# Autodesk Inventor assembly: Box Arm
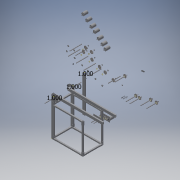
[picture p0: Inventor's stored thumbnail of the model, 180x180]
Saved by Autodesk Inventor 2018 (Build 220112000, 112)
## iProperties
Created: 2019-01-16
Part Number: Box Arm
Document SubType Name: Assembly
Designer: Gabriel
Author: Gabriel
## Documents named in this file (20)
- C:\Users\Gabriel\Documents\GitHub\2019CAD\Drivebase Box Arm\Box Arm.iam
- C:\Users\Gabriel\Documents\GitHub\2019CAD\Drivebase Box Arm\30in 1x1 Beam.ipt
- C:\Users\Gabriel\Documents\GitHub\2019CAD\Drivebase Box Arm\25in 1x1 Beam.ipt
- C:\Users\Gabriel\Documents\GitHub\2019CAD\Drivebase Box Arm\17in 1x1 Beam.ipt
- C:\Users\Gabriel\Documents\GitHub\2019CAD\Drivebase Box Arm\23in 1x1 Beam.ipt
- C:\Users\Gabriel\Documents\GitHub\2019CAD\Drivebase Box Arm\L gusset.ipt
- C:\Users\Gabriel\Documents\GitHub\2019CAD\Drivebase Box Arm\34.48in Arm Bea.ipt
- C:\Users\Gabriel\Documents\GitHub\2019CAD\Drivebase Box Arm\0_500_ID_x_1_125_OD_x_0_313_WD_Flanged_Bearing_217-2731.ipt
- C:\Users\Gabriel\Documents\GitHub\2019CAD\Drivebase Box Arm\_72t_Aluminum_Plate_Sprocket_25_Chain_1-1_8_Bearing_Bore_217-2627.ipt
- C:\Users\Gabriel\Documents\GitHub\2019CAD\Drivebase Box Arm\Hex Hub.ipt
- C:\Users\Gabriel\Documents\GitHub\2019CAD\Drivebase Box Arm\0.5in Hex Shaft.ipt
- C:\Users\Gabriel\Documents\GitHub\2019CAD\Drivebase Box Arm\half_inch_collar.ipt
- C:\Users\Gabriel\Documents\GitHub\2019CAD\Drivebase Box Arm\1_2_Acetal_Spacer_-_1_2_Hex_217-3261.ipt
- C:\Users\Gabriel\Documents\GitHub\2019CAD\Drivebase Box Arm\_16t_Aluminum_Hub_Sprocket_25_Chain_1_2_Hex_Bore_217-2642.ipt
- C:\Users\Gabriel\Documents\GitHub\2019CAD\Drivebase Box Arm\18t_Aluminum_Spur_Gear_20_DP_1_2_Hex_Bore_217-3209.ipt
- C:\Users\Gabriel\Documents\GitHub\2019CAD\Drivebase Box Arm\am-0150 Toughbox Large Output Gear.ipt
- C:\Users\Gabriel\Documents\GitHub\2019CAD\Drivebase Box Arm\Mini_CIM_Motor_217-3371.ipt
- C:\Users\Gabriel\Documents\GitHub\2019CAD\Drivebase Box Arm\9T_Steel_Spur_Gear_20_DP_10T_Center_Distance_CIM_Motor_217-6335.ipt
- C:\Users\Gabriel\Documents\GitHub\2019CAD\Drivebase Box Arm\ARm Gearbox Plate.ipt
- C:\Users\Gabriel\Documents\GitHub\2019CAD\Drivebase Box Arm\1_16_Acetal_Spacer_-_1_2_Hex_217-3257.ipt
## Components (159 placed, 19 different names)
1. 30in 1x1 Beam:1 — Mate:13, Mate:14, Mate:37, Mate:38, Mate:74, Mate:75, Mate:83, Mate:84, Mate:98, Mate:99, Mate:101, Mate:102, Mate:103, Mate:104
2. 30in 1x1 Beam:2 — Mate:11, Mate:12, Mate:39, Mate:40, Mate:73, Mate:76, Mate:86, Mate:87, Mate:95, Mate:96, Mate:105, Mate:106, Mate:107, Mate:108
3. 25in 1x1 Beam:1 — Mate:57, Mate:58, Mate:59, Mate:60, Mate:65, Mate:66, Mate:90, Mate:91
4. 25in 1x1 Beam:2 — Mate:61, Mate:62, Mate:63, Mate:64, Mate:67, Mate:68, Mate:93, Mate:94
5. 25in 1x1 Beam:3 — Mate:29, Mate:30, Mate:53, Mate:54, Mate:97
6. 25in 1x1 Beam:4 — Mate:31, Mate:32, Mate:55, Mate:56, Mate:100
7. 17in 1x1 Beam:1 — Mate:69, Mate:70, Mate:71, Mate:72
8. 17in 1x1 Beam:2 — Mate:21, Mate:22, Mate:23, Mate:24
9. 23in 1x1 Beam:1 — Mate:43, Mate:44, Mate:49, Mate:50, Mate:88, Mate:92
10. 23in 1x1 Beam:2 — Mate:47, Mate:48, Mate:51, Mate:52, Mate:85, Mate:89
11. L gusset:1 — Mate:53, Mate:54, Mate:63, Mate:64
12. L gusset:4 — Mate:49, Mate:50, Mate:61, Mate:62
13. L gusset:5 — Mate:51, Mate:52, Mate:57, Mate:58
14. L gusset:7 — Mate:11, Mate:12, Mate:23, Mate:24
15. L gusset:9 — Mate:13, Mate:14, Mate:21, Mate:22
16. L gusset:11 — Mate:31, Mate:32, Mate:74, Mate:75
17. L gusset:12 — Mate:29, Mate:30, Mate:73, Mate:76
18. L gusset:13 — Mate:43, Mate:44
19. L gusset:14 — Mate:47, Mate:48
20. L gusset:15 — Mate:39, Mate:40, Mate:77, Mate:80
21. L gusset:16 — Mate:37, Mate:38, Mate:78, Mate:79
22. L gusset:17 — Mate:55, Mate:56, Mate:59, Mate:60
23. L gusset:18 — Mate:67, Mate:68, Mate:69, Mate:70
24. L gusset:19 — Mate:65, Mate:66, Mate:71, Mate:72
25. 17in 1x1 Beam:3 — Mate:77, Mate:78, Mate:79, Mate:80
26. 34.48in Arm Bea:2 — Mate:109, Mate:110, Mate:145
27. 0_500_ID_x_1_125_OD_x_0_313_WD_Flanged_Bearing_217-2731:1 — Mate:103, Mate:104, Mate:139, Mate:140, Mate:149
28. 0_500_ID_x_1_125_OD_x_0_313_WD_Flanged_Bearing_217-2731:2 — Mate:107, Mate:108, Mate:126, Mate:152
29. 0_500_ID_x_1_125_OD_x_0_313_WD_Flanged_Bearing_217-2731:3
30. 0_500_ID_x_1_125_OD_x_0_313_WD_Flanged_Bearing_217-2731:5 — Mate:101, Mate:102, Mate:143
31. 0_500_ID_x_1_125_OD_x_0_313_WD_Flanged_Bearing_217-2731:8 — Mate:105, Mate:106, Mate:122
32. L gusset:20 — Mate:92, Mate:93, Mate:94
33. L gusset:21 — Mate:89, Mate:90, Mate:91
34. L gusset:22 — Mate:98, Mate:99, Mate:100
35. L gusset:23 — Mate:95, Mate:96, Mate:97
36. L gusset:24 — Mate:83, Mate:84, Mate:85
37. L gusset:25 — Mate:86, Mate:87, Mate:88
38. _72t_Aluminum_Plate_Sprocket_25_Chain_1-1_8_Bearing_Bore_217-2627:2 — Mate:120, Mate:121, Mate:138
39. Hex Hub:2 — Mate:109, Mate:110, Mate:111, Mate:112, Mate:113, Mate:114, Mate:115
40. Hex Hub:3 — Mate:116, Mate:117, Mate:118, Mate:120, Mate:121, Mate:122, Mate:138
41. 0.5in Hex Shaft:2 — Mate:114, Mate:115, Mate:116, Mate:117, Mate:123, Mate:124, Mate:125, Mate:150, Mate:151
42. half_inch_collar:1 — Mate:145
43. half_inch_collar:2 — Mate:146
44. half_inch_collar:4 — Mate:127
45. 1_2_Acetal_Spacer_-_1_2_Hex_217-3261:1 — Mate:123, Mate:124, Mate:125, Mate:126, Mate:127
46. 1_2_Acetal_Spacer_-_1_2_Hex_217-3261:3 — Mate:111, Mate:112, Mate:113, Mate:118
47. 34.48in Arm Bea:3 — Mate:128, Mate:146
48. _72t_Aluminum_Plate_Sprocket_25_Chain_1-1_8_Bearing_Bore_217-2627:3 — Mate:137
49. Hex Hub:4 — Mate:134, Mate:135, Mate:136, Mate:137, Mate:139, Mate:140
50. Hex Hub:5 — Mate:128, Mate:129, Mate:130, Mate:133
51. 0.5in Hex Shaft:3 — Mate:129, Mate:130, Mate:131, Mate:132, Mate:134, Mate:135, Mate:141, Mate:142, Mate:147, Mate:148
52. half_inch_collar:5 — Mate:144
53. 1_2_Acetal_Spacer_-_1_2_Hex_217-3261:7 — Mate:141, Mate:142, Mate:143, Mate:144
54. 1_2_Acetal_Spacer_-_1_2_Hex_217-3261:8 — Mate:131, Mate:132, Mate:133, Mate:136
55. 1_2_Acetal_Spacer_-_1_2_Hex_217-3261:9 — Mate:147, Mate:148, Mate:149
56. 1_2_Acetal_Spacer_-_1_2_Hex_217-3261:10 — Mate:150, Mate:151, Mate:152
57. 30in 1x1 Beam:3
58. _16t_Aluminum_Hub_Sprocket_25_Chain_1_2_Hex_Bore_217-2642:1
59. 0.5in Hex Shaft:4
60. 18t_Aluminum_Spur_Gear_20_DP_1_2_Hex_Bore_217-3209:1
61. am-0150 Toughbox Large Output Gear:1
62. half_inch_collar:6
63. Mini_CIM_Motor_217-3371:1
64. _16t_Aluminum_Hub_Sprocket_25_Chain_1_2_Hex_Bore_217-2642:2
65. 0.5in Hex Shaft:5
66. 18t_Aluminum_Spur_Gear_20_DP_1_2_Hex_Bore_217-3209:2
67. am-0150 Toughbox Large Output Gear:2
68. half_inch_collar:7
69. Mini_CIM_Motor_217-3371:2 — Mate:165, Mate:166, Mate:167, Mate:168
70. _16t_Aluminum_Hub_Sprocket_25_Chain_1_2_Hex_Bore_217-2642:3
71. 0.5in Hex Shaft:6 — Mate:169, Mate:170, Mate:171, Mate:172, Mate:173
72. 18t_Aluminum_Spur_Gear_20_DP_1_2_Hex_Bore_217-3209:3 — Mate:172, Mate:173, Mate:174
73. am-0150 Toughbox Large Output Gear:3 — Mate:169, Mate:170, Mate:171, Mate:174
74. half_inch_collar:8
75. Mini_CIM_Motor_217-3371:3
76. _16t_Aluminum_Hub_Sprocket_25_Chain_1_2_Hex_Bore_217-2642:4
77. half_inch_collar:9
78. Mini_CIM_Motor_217-3371:4
79. _16t_Aluminum_Hub_Sprocket_25_Chain_1_2_Hex_Bore_217-2642:5
80. 0.5in Hex Shaft:8
81. 18t_Aluminum_Spur_Gear_20_DP_1_2_Hex_Bore_217-3209:5
82. am-0150 Toughbox Large Output Gear:5
83. half_inch_collar:10
84. Mini_CIM_Motor_217-3371:5
85. _16t_Aluminum_Hub_Sprocket_25_Chain_1_2_Hex_Bore_217-2642:6
86. 0.5in Hex Shaft:9
87. 18t_Aluminum_Spur_Gear_20_DP_1_2_Hex_Bore_217-3209:6
88. am-0150 Toughbox Large Output Gear:6
89. half_inch_collar:11
90. Mini_CIM_Motor_217-3371:6
91. _16t_Aluminum_Hub_Sprocket_25_Chain_1_2_Hex_Bore_217-2642:7
92. 0.5in Hex Shaft:10
93. 18t_Aluminum_Spur_Gear_20_DP_1_2_Hex_Bore_217-3209:7
94. am-0150 Toughbox Large Output Gear:7
95. half_inch_collar:12
96. Mini_CIM_Motor_217-3371:7
97. _16t_Aluminum_Hub_Sprocket_25_Chain_1_2_Hex_Bore_217-2642:8
98. 0.5in Hex Shaft:11
99. 18t_Aluminum_Spur_Gear_20_DP_1_2_Hex_Bore_217-3209:8
100. am-0150 Toughbox Large Output Gear:8
101. half_inch_collar:13
102. Mini_CIM_Motor_217-3371:8
103. 9T_Steel_Spur_Gear_20_DP_10T_Center_Distance_CIM_Motor_217-6335:1
104. 9T_Steel_Spur_Gear_20_DP_10T_Center_Distance_CIM_Motor_217-6335:2 — Mate:167, Mate:168
105. ARm Gearbox Plate:1 — Mate:159, Mate:160, Mate:161, Mate:162, Mate:163, Mate:164
106. ARm Gearbox Plate:2 — Mate:153, Mate:154, Mate:155, Mate:156, Mate:157, Mate:158, Mate:165, Mate:166
107. 0_500_ID_x_1_125_OD_x_0_313_WD_Flanged_Bearing_217-2731:9 — Mate:153, Mate:156, Mate:200, Mate:201
108. 0_500_ID_x_1_125_OD_x_0_313_WD_Flanged_Bearing_217-2731:10 — Mate:155, Mate:158, Mate:272
109. 0_500_ID_x_1_125_OD_x_0_313_WD_Flanged_Bearing_217-2731:11 — Mate:154, Mate:157, Mate:241
110. 0_500_ID_x_1_125_OD_x_0_313_WD_Flanged_Bearing_217-2731:12 — Mate:160, Mate:163
111. 0_500_ID_x_1_125_OD_x_0_313_WD_Flanged_Bearing_217-2731:13 — Mate:159, Mate:164
112. 0_500_ID_x_1_125_OD_x_0_313_WD_Flanged_Bearing_217-2731:14 — Mate:161, Mate:162
113. 0.5in Hex Shaft:12 — Mate:188, Mate:189
114. 18t_Aluminum_Spur_Gear_20_DP_1_2_Hex_Bore_217-3209:9
115. am-0150 Toughbox Large Output Gear:9 — Mate:190
116. 1_16_Acetal_Spacer_-_1_2_Hex_217-3257:1
117. 1_16_Acetal_Spacer_-_1_2_Hex_217-3257:2 — Mate:188, Mate:189, Mate:190
118. 1_16_Acetal_Spacer_-_1_2_Hex_217-3257:3
119. 1_16_Acetal_Spacer_-_1_2_Hex_217-3257:4
120. 1_16_Acetal_Spacer_-_1_2_Hex_217-3257:5
121. 1_16_Acetal_Spacer_-_1_2_Hex_217-3257:6
122. 1_16_Acetal_Spacer_-_1_2_Hex_217-3257:7
123. 1_16_Acetal_Spacer_-_1_2_Hex_217-3257:8
124. 1_16_Acetal_Spacer_-_1_2_Hex_217-3257:9
125. 1_16_Acetal_Spacer_-_1_2_Hex_217-3257:10
126. 0.5in Hex Shaft:13 — Mate:199
127. 18t_Aluminum_Spur_Gear_20_DP_1_2_Hex_Bore_217-3209:10 — Mate:199
128. am-0150 Toughbox Large Output Gear:10
129. 1_16_Acetal_Spacer_-_1_2_Hex_217-3257:11 — Mate:200, Mate:201
130. 0.5in Hex Shaft:14 — Mate:210, Mate:211, Mate:212
131. 18t_Aluminum_Spur_Gear_20_DP_1_2_Hex_Bore_217-3209:11 — Mate:210
132. am-0150 Toughbox Large Output Gear:11 — Mate:240
133. 1_2_Acetal_Spacer_-_1_2_Hex_217-3261:11
134. 1_2_Acetal_Spacer_-_1_2_Hex_217-3261:12 — Mate:242, Mate:243, Mate:244, Mate:247
135. 1_2_Acetal_Spacer_-_1_2_Hex_217-3261:13
136. 1_2_Acetal_Spacer_-_1_2_Hex_217-3261:14 — Mate:245, Mate:246, Mate:247, Mate:272
137. 1_2_Acetal_Spacer_-_1_2_Hex_217-3261:15
138. 1_2_Acetal_Spacer_-_1_2_Hex_217-3261:16 — Mate:211, Mate:212, Mate:240, Mate:241
139. 0.5in Hex Shaft:15 — Mate:242, Mate:243, Mate:245, Mate:246
140. 18t_Aluminum_Spur_Gear_20_DP_1_2_Hex_Bore_217-3209:12
141. am-0150 Toughbox Large Output Gear:12 — Mate:244
142. 0.5in Hex Shaft:16
143. 18t_Aluminum_Spur_Gear_20_DP_1_2_Hex_Bore_217-3209:13
144. am-0150 Toughbox Large Output Gear:13
145. 1_16_Acetal_Spacer_-_1_2_Hex_217-3257:14
146. 0.5in Hex Shaft:17
147. 18t_Aluminum_Spur_Gear_20_DP_1_2_Hex_Bore_217-3209:14
148. am-0150 Toughbox Large Output Gear:14
149. 1_16_Acetal_Spacer_-_1_2_Hex_217-3257:15
150. 1_2_Acetal_Spacer_-_1_2_Hex_217-3261:17
151. 1_2_Acetal_Spacer_-_1_2_Hex_217-3261:18
152. 0.5in Hex Shaft:18
153. 18t_Aluminum_Spur_Gear_20_DP_1_2_Hex_Bore_217-3209:15
154. am-0150 Toughbox Large Output Gear:15
155. 1_2_Acetal_Spacer_-_1_2_Hex_217-3261:19
156. 1_2_Acetal_Spacer_-_1_2_Hex_217-3261:20
157. 0.5in Hex Shaft:19
158. 18t_Aluminum_Spur_Gear_20_DP_1_2_Hex_Bore_217-3209:16
159. am-0150 Toughbox Large Output Gear:16
## Relationships (227: Mate 227)
- Mate:11: 30in 1x1 Beam:2 ↔ L gusset:7
- Mate:12: 30in 1x1 Beam:2 ↔ L gusset:7
- Mate:13: 30in 1x1 Beam:1 ↔ L gusset:9
- Mate:14: 30in 1x1 Beam:1 ↔ L gusset:9
- Mate:21: 17in 1x1 Beam:2 ↔ L gusset:9
- Mate:22: 17in 1x1 Beam:2 ↔ L gusset:9
- Mate:23: 17in 1x1 Beam:2 ↔ L gusset:7
- Mate:24: 17in 1x1 Beam:2 ↔ L gusset:7
- Mate:29: 25in 1x1 Beam:3 ↔ L gusset:12
- Mate:30: 25in 1x1 Beam:3 ↔ L gusset:12
- Mate:31: 25in 1x1 Beam:4 ↔ L gusset:11
- Mate:32: 25in 1x1 Beam:4 ↔ L gusset:11
- Mate:37: 30in 1x1 Beam:1 ↔ L gusset:16
- Mate:38: 30in 1x1 Beam:1 ↔ L gusset:16
- Mate:39: 30in 1x1 Beam:2 ↔ L gusset:15
- Mate:40: 30in 1x1 Beam:2 ↔ L gusset:15
- Mate:43: 23in 1x1 Beam:1 ↔ L gusset:13
- Mate:44: 23in 1x1 Beam:1 ↔ L gusset:13
- Mate:47: 23in 1x1 Beam:2 ↔ L gusset:14
- Mate:48: 23in 1x1 Beam:2 ↔ L gusset:14
- Mate:49: 23in 1x1 Beam:1 ↔ L gusset:4
- Mate:50: 23in 1x1 Beam:1 ↔ L gusset:4
- Mate:51: 23in 1x1 Beam:2 ↔ L gusset:5
- Mate:52: 23in 1x1 Beam:2 ↔ L gusset:5
- Mate:53: 25in 1x1 Beam:3 ↔ L gusset:1
- Mate:54: 25in 1x1 Beam:3 ↔ L gusset:1
- Mate:55: 25in 1x1 Beam:4 ↔ L gusset:17
- Mate:56: 25in 1x1 Beam:4 ↔ L gusset:17
- Mate:57: 25in 1x1 Beam:1 ↔ L gusset:5
- Mate:58: 25in 1x1 Beam:1 ↔ L gusset:5
- Mate:59: 25in 1x1 Beam:1 ↔ L gusset:17
- Mate:60: 25in 1x1 Beam:1 ↔ L gusset:17
- Mate:61: 25in 1x1 Beam:2 ↔ L gusset:4
- Mate:62: 25in 1x1 Beam:2 ↔ L gusset:4
- Mate:63: 25in 1x1 Beam:2 ↔ L gusset:1
- Mate:64: 25in 1x1 Beam:2 ↔ L gusset:1
- Mate:65: 25in 1x1 Beam:1 ↔ L gusset:19
- Mate:66: 25in 1x1 Beam:1 ↔ L gusset:19
- Mate:67: 25in 1x1 Beam:2 ↔ L gusset:18
- Mate:68: 25in 1x1 Beam:2 ↔ L gusset:18
- Mate:69: 17in 1x1 Beam:1 ↔ L gusset:18
- Mate:70: 17in 1x1 Beam:1 ↔ L gusset:18
- Mate:71: 17in 1x1 Beam:1 ↔ L gusset:19
- Mate:72: 17in 1x1 Beam:1 ↔ L gusset:19
- Mate:73: 30in 1x1 Beam:2 ↔ L gusset:12
- Mate:74: 30in 1x1 Beam:1 ↔ L gusset:11
- Mate:75: 30in 1x1 Beam:1 ↔ L gusset:11
- Mate:76: 30in 1x1 Beam:2 ↔ L gusset:12
- Mate:77: L gusset:15 ↔ 17in 1x1 Beam:3
- Mate:78: L gusset:16 ↔ 17in 1x1 Beam:3
- Mate:79: L gusset:16 ↔ 17in 1x1 Beam:3
- Mate:80: L gusset:15 ↔ 17in 1x1 Beam:3
- Mate:83: 30in 1x1 Beam:1 ↔ L gusset:24
- Mate:84: 30in 1x1 Beam:1 ↔ L gusset:24
- Mate:85: 23in 1x1 Beam:2 ↔ L gusset:24
- Mate:86: 30in 1x1 Beam:2 ↔ L gusset:25
- Mate:87: 30in 1x1 Beam:2 ↔ L gusset:25
- Mate:88: 23in 1x1 Beam:1 ↔ L gusset:25
- Mate:89: 23in 1x1 Beam:2 ↔ L gusset:21
- Mate:90: 25in 1x1 Beam:1 ↔ L gusset:21
- Mate:91: 25in 1x1 Beam:1 ↔ L gusset:21
- Mate:92: 23in 1x1 Beam:1 ↔ L gusset:20
- Mate:93: 25in 1x1 Beam:2 ↔ L gusset:20
- Mate:94: 25in 1x1 Beam:2 ↔ L gusset:20
- Mate:95: 30in 1x1 Beam:2 ↔ L gusset:23
- Mate:96: 30in 1x1 Beam:2 ↔ L gusset:23
- Mate:97: 25in 1x1 Beam:3 ↔ L gusset:23
- Mate:98: 30in 1x1 Beam:1 ↔ L gusset:22
- Mate:99: 30in 1x1 Beam:1 ↔ L gusset:22
- Mate:100: 25in 1x1 Beam:4 ↔ L gusset:22
- Mate:101: 30in 1x1 Beam:1 ↔ 0_500_ID_x_1_125_OD_x_0_313_WD_Flanged_Bearing_217-2731:5
- Mate:102: 30in 1x1 Beam:1 ↔ 0_500_ID_x_1_125_OD_x_0_313_WD_Flanged_Bearing_217-2731:5
- Mate:103: 30in 1x1 Beam:1 ↔ 0_500_ID_x_1_125_OD_x_0_313_WD_Flanged_Bearing_217-2731:1
- Mate:104: 30in 1x1 Beam:1 ↔ 0_500_ID_x_1_125_OD_x_0_313_WD_Flanged_Bearing_217-2731:1
- Mate:105: 30in 1x1 Beam:2 ↔ 0_500_ID_x_1_125_OD_x_0_313_WD_Flanged_Bearing_217-2731:8
- Mate:106: 30in 1x1 Beam:2 ↔ 0_500_ID_x_1_125_OD_x_0_313_WD_Flanged_Bearing_217-2731:8
- Mate:107: 30in 1x1 Beam:2 ↔ 0_500_ID_x_1_125_OD_x_0_313_WD_Flanged_Bearing_217-2731:2
- Mate:108: 30in 1x1 Beam:2 ↔ 0_500_ID_x_1_125_OD_x_0_313_WD_Flanged_Bearing_217-2731:2
- Mate:109: 34.48in Arm Bea:2 ↔ Hex Hub:2
- Mate:110: 34.48in Arm Bea:2 ↔ Hex Hub:2
- Mate:111: Hex Hub:2 ↔ 1_2_Acetal_Spacer_-_1_2_Hex_217-3261:3
- Mate:112: Hex Hub:2 ↔ 1_2_Acetal_Spacer_-_1_2_Hex_217-3261:3
- Mate:113: Hex Hub:2 ↔ 1_2_Acetal_Spacer_-_1_2_Hex_217-3261:3
- Mate:114: Hex Hub:2 ↔ 0.5in Hex Shaft:2
- Mate:115: Hex Hub:2 ↔ 0.5in Hex Shaft:2
- Mate:116: Hex Hub:3 ↔ 0.5in Hex Shaft:2
- Mate:117: Hex Hub:3 ↔ 0.5in Hex Shaft:2
- Mate:118: Hex Hub:3 ↔ 1_2_Acetal_Spacer_-_1_2_Hex_217-3261:3
- Mate:120: _72t_Aluminum_Plate_Sprocket_25_Chain_1-1_8_Bearing_Bore_217-2627:2 ↔ Hex Hub:3
- Mate:121: _72t_Aluminum_Plate_Sprocket_25_Chain_1-1_8_Bearing_Bore_217-2627:2 ↔ Hex Hub:3
- Mate:122: 0_500_ID_x_1_125_OD_x_0_313_WD_Flanged_Bearing_217-2731:8 ↔ Hex Hub:3
- Mate:123: 0.5in Hex Shaft:2 ↔ 1_2_Acetal_Spacer_-_1_2_Hex_217-3261:1
- Mate:124: 0.5in Hex Shaft:2 ↔ 1_2_Acetal_Spacer_-_1_2_Hex_217-3261:1
- Mate:125: 0.5in Hex Shaft:2 ↔ 1_2_Acetal_Spacer_-_1_2_Hex_217-3261:1
- Mate:126: 0_500_ID_x_1_125_OD_x_0_313_WD_Flanged_Bearing_217-2731:2 ↔ 1_2_Acetal_Spacer_-_1_2_Hex_217-3261:1
- Mate:127: half_inch_collar:4 ↔ 1_2_Acetal_Spacer_-_1_2_Hex_217-3261:1
- Mate:128: 34.48in Arm Bea:3 ↔ Hex Hub:5
- Mate:129: Hex Hub:5 ↔ 0.5in Hex Shaft:3
- Mate:130: Hex Hub:5 ↔ 0.5in Hex Shaft:3
- Mate:131: 0.5in Hex Shaft:3 ↔ 1_2_Acetal_Spacer_-_1_2_Hex_217-3261:8
- Mate:132: 0.5in Hex Shaft:3 ↔ 1_2_Acetal_Spacer_-_1_2_Hex_217-3261:8
- Mate:133: Hex Hub:5 ↔ 1_2_Acetal_Spacer_-_1_2_Hex_217-3261:8
- Mate:134: Hex Hub:4 ↔ 0.5in Hex Shaft:3
- Mate:135: Hex Hub:4 ↔ 0.5in Hex Shaft:3
- Mate:136: Hex Hub:4 ↔ 1_2_Acetal_Spacer_-_1_2_Hex_217-3261:8
- Mate:137: _72t_Aluminum_Plate_Sprocket_25_Chain_1-1_8_Bearing_Bore_217-2627:3 ↔ Hex Hub:4
- Mate:138: _72t_Aluminum_Plate_Sprocket_25_Chain_1-1_8_Bearing_Bore_217-2627:2 ↔ Hex Hub:3
- Mate:139: 0_500_ID_x_1_125_OD_x_0_313_WD_Flanged_Bearing_217-2731:1 ↔ Hex Hub:4
- Mate:140: 0_500_ID_x_1_125_OD_x_0_313_WD_Flanged_Bearing_217-2731:1 ↔ Hex Hub:4
- Mate:141: 0.5in Hex Shaft:3 ↔ 1_2_Acetal_Spacer_-_1_2_Hex_217-3261:7
- Mate:142: 0.5in Hex Shaft:3 ↔ 1_2_Acetal_Spacer_-_1_2_Hex_217-3261:7
- Mate:143: 0_500_ID_x_1_125_OD_x_0_313_WD_Flanged_Bearing_217-2731:5 ↔ 1_2_Acetal_Spacer_-_1_2_Hex_217-3261:7
- Mate:144: half_inch_collar:5 ↔ 1_2_Acetal_Spacer_-_1_2_Hex_217-3261:7
- Mate:145: 34.48in Arm Bea:2 ↔ half_inch_collar:1
- Mate:146: half_inch_collar:2 ↔ 34.48in Arm Bea:3
- Mate:147: 0.5in Hex Shaft:3 ↔ 1_2_Acetal_Spacer_-_1_2_Hex_217-3261:9
- Mate:148: 0.5in Hex Shaft:3 ↔ 1_2_Acetal_Spacer_-_1_2_Hex_217-3261:9
- Mate:149: 0_500_ID_x_1_125_OD_x_0_313_WD_Flanged_Bearing_217-2731:1 ↔ 1_2_Acetal_Spacer_-_1_2_Hex_217-3261:9
- Mate:150: 0.5in Hex Shaft:2 ↔ 1_2_Acetal_Spacer_-_1_2_Hex_217-3261:10
- Mate:151: 0.5in Hex Shaft:2 ↔ 1_2_Acetal_Spacer_-_1_2_Hex_217-3261:10
- Mate:152: 0_500_ID_x_1_125_OD_x_0_313_WD_Flanged_Bearing_217-2731:2 ↔ 1_2_Acetal_Spacer_-_1_2_Hex_217-3261:10
- Mate:153: ARm Gearbox Plate:2 ↔ 0_500_ID_x_1_125_OD_x_0_313_WD_Flanged_Bearing_217-2731:9
- Mate:154: ARm Gearbox Plate:2 ↔ 0_500_ID_x_1_125_OD_x_0_313_WD_Flanged_Bearing_217-2731:11
- Mate:155: ARm Gearbox Plate:2 ↔ 0_500_ID_x_1_125_OD_x_0_313_WD_Flanged_Bearing_217-2731:10
- Mate:156: ARm Gearbox Plate:2 ↔ 0_500_ID_x_1_125_OD_x_0_313_WD_Flanged_Bearing_217-2731:9
- Mate:157: ARm Gearbox Plate:2 ↔ 0_500_ID_x_1_125_OD_x_0_313_WD_Flanged_Bearing_217-2731:11
- Mate:158: ARm Gearbox Plate:2 ↔ 0_500_ID_x_1_125_OD_x_0_313_WD_Flanged_Bearing_217-2731:10
- Mate:159: ARm Gearbox Plate:1 ↔ 0_500_ID_x_1_125_OD_x_0_313_WD_Flanged_Bearing_217-2731:13
- Mate:160: ARm Gearbox Plate:1 ↔ 0_500_ID_x_1_125_OD_x_0_313_WD_Flanged_Bearing_217-2731:12
- Mate:161: ARm Gearbox Plate:1 ↔ 0_500_ID_x_1_125_OD_x_0_313_WD_Flanged_Bearing_217-2731:14
- Mate:162: ARm Gearbox Plate:1 ↔ 0_500_ID_x_1_125_OD_x_0_313_WD_Flanged_Bearing_217-2731:14
- Mate:163: ARm Gearbox Plate:1 ↔ 0_500_ID_x_1_125_OD_x_0_313_WD_Flanged_Bearing_217-2731:12
- Mate:164: ARm Gearbox Plate:1 ↔ 0_500_ID_x_1_125_OD_x_0_313_WD_Flanged_Bearing_217-2731:13
- Mate:165: Mini_CIM_Motor_217-3371:2 ↔ ARm Gearbox Plate:2
- Mate:166: Mini_CIM_Motor_217-3371:2 ↔ ARm Gearbox Plate:2
- Mate:167: Mini_CIM_Motor_217-3371:2 ↔ 9T_Steel_Spur_Gear_20_DP_10T_Center_Distance_CIM_Motor_217-6335:2
- Mate:168: Mini_CIM_Motor_217-3371:2 ↔ 9T_Steel_Spur_Gear_20_DP_10T_Center_Distance_CIM_Motor_217-6335:2
- Mate:169: 0.5in Hex Shaft:6 ↔ am-0150 Toughbox Large Output Gear:3
- Mate:170: 0.5in Hex Shaft:6 ↔ am-0150 Toughbox Large Output Gear:3
- Mate:171: 0.5in Hex Shaft:6 ↔ am-0150 Toughbox Large Output Gear:3
- Mate:172: 0.5in Hex Shaft:6 ↔ 18t_Aluminum_Spur_Gear_20_DP_1_2_Hex_Bore_217-3209:3
- Mate:173: 0.5in Hex Shaft:6 ↔ 18t_Aluminum_Spur_Gear_20_DP_1_2_Hex_Bore_217-3209:3
- Mate:174: 18t_Aluminum_Spur_Gear_20_DP_1_2_Hex_Bore_217-3209:3 ↔ am-0150 Toughbox Large Output Gear:3
- [Mate]: 0.5in Hex Shaft:12 ↔ am-0150 Toughbox Large Output Gear:9
- [Mate]: 0.5in Hex Shaft:12 ↔ am-0150 Toughbox Large Output Gear:9
- [Mate]: 0.5in Hex Shaft:12 ↔ am-0150 Toughbox Large Output Gear:9
- [Mate]: 0.5in Hex Shaft:12 ↔ 18t_Aluminum_Spur_Gear_20_DP_1_2_Hex_Bore_217-3209:9
- [Mate]: 18t_Aluminum_Spur_Gear_20_DP_1_2_Hex_Bore_217-3209:9 ↔ am-0150 Toughbox Large Output Gear:9
- Mate:188: 0.5in Hex Shaft:12 ↔ 1_16_Acetal_Spacer_-_1_2_Hex_217-3257:2
- Mate:189: 0.5in Hex Shaft:12 ↔ 1_16_Acetal_Spacer_-_1_2_Hex_217-3257:2
- Mate:190: am-0150 Toughbox Large Output Gear:9 ↔ 1_16_Acetal_Spacer_-_1_2_Hex_217-3257:2
- [Mate]: 0.5in Hex Shaft:13 ↔ am-0150 Toughbox Large Output Gear:10
- [Mate]: 0.5in Hex Shaft:13 ↔ am-0150 Toughbox Large Output Gear:10
- [Mate]: 0.5in Hex Shaft:13 ↔ am-0150 Toughbox Large Output Gear:10
- [Mate]: 0.5in Hex Shaft:13 ↔ 18t_Aluminum_Spur_Gear_20_DP_1_2_Hex_Bore_217-3209:10
- [Mate]: 18t_Aluminum_Spur_Gear_20_DP_1_2_Hex_Bore_217-3209:10 ↔ am-0150 Toughbox Large Output Gear:10
- [Mate]: 0.5in Hex Shaft:13 ↔ 1_16_Acetal_Spacer_-_1_2_Hex_217-3257:11
- [Mate]: 0.5in Hex Shaft:13 ↔ 1_16_Acetal_Spacer_-_1_2_Hex_217-3257:11
- [Mate]: am-0150 Toughbox Large Output Gear:10 ↔ 1_16_Acetal_Spacer_-_1_2_Hex_217-3257:11
- Mate:199: 0.5in Hex Shaft:13 ↔ 18t_Aluminum_Spur_Gear_20_DP_1_2_Hex_Bore_217-3209:10
- Mate:200: 0_500_ID_x_1_125_OD_x_0_313_WD_Flanged_Bearing_217-2731:9 ↔ 1_16_Acetal_Spacer_-_1_2_Hex_217-3257:11
- Mate:201: 0_500_ID_x_1_125_OD_x_0_313_WD_Flanged_Bearing_217-2731:9 ↔ 1_16_Acetal_Spacer_-_1_2_Hex_217-3257:11
- [Mate]: 0.5in Hex Shaft:14 ↔ am-0150 Toughbox Large Output Gear:11
- [Mate]: 0.5in Hex Shaft:14 ↔ am-0150 Toughbox Large Output Gear:11
- [Mate]: 0.5in Hex Shaft:14 ↔ am-0150 Toughbox Large Output Gear:11
- [Mate]: 0.5in Hex Shaft:14 ↔ 18t_Aluminum_Spur_Gear_20_DP_1_2_Hex_Bore_217-3209:11
- [Mate]: 18t_Aluminum_Spur_Gear_20_DP_1_2_Hex_Bore_217-3209:11 ↔ am-0150 Toughbox Large Output Gear:11
- Mate:210: 0.5in Hex Shaft:14 ↔ 18t_Aluminum_Spur_Gear_20_DP_1_2_Hex_Bore_217-3209:11
- Mate:211: 0.5in Hex Shaft:14 ↔ 1_2_Acetal_Spacer_-_1_2_Hex_217-3261:16
- Mate:212: 0.5in Hex Shaft:14 ↔ 1_2_Acetal_Spacer_-_1_2_Hex_217-3261:16
- [Mate]: 0.5in Hex Shaft:15 ↔ am-0150 Toughbox Large Output Gear:12
- [Mate]: 0.5in Hex Shaft:15 ↔ am-0150 Toughbox Large Output Gear:12
- [Mate]: 0.5in Hex Shaft:15 ↔ am-0150 Toughbox Large Output Gear:12
- [Mate]: 0.5in Hex Shaft:15 ↔ 18t_Aluminum_Spur_Gear_20_DP_1_2_Hex_Bore_217-3209:12
- [Mate]: 18t_Aluminum_Spur_Gear_20_DP_1_2_Hex_Bore_217-3209:12 ↔ am-0150 Toughbox Large Output Gear:12
- [Mate]: 0.5in Hex Shaft:15 ↔ 18t_Aluminum_Spur_Gear_20_DP_1_2_Hex_Bore_217-3209:12
- [Mate]: 0.5in Hex Shaft:16 ↔ am-0150 Toughbox Large Output Gear:13
- [Mate]: 0.5in Hex Shaft:16 ↔ am-0150 Toughbox Large Output Gear:13
- [Mate]: 0.5in Hex Shaft:16 ↔ am-0150 Toughbox Large Output Gear:13
- [Mate]: 0.5in Hex Shaft:16 ↔ 18t_Aluminum_Spur_Gear_20_DP_1_2_Hex_Bore_217-3209:13
- [Mate]: 18t_Aluminum_Spur_Gear_20_DP_1_2_Hex_Bore_217-3209:13 ↔ am-0150 Toughbox Large Output Gear:13
- [Mate]: 0.5in Hex Shaft:16 ↔ 1_16_Acetal_Spacer_-_1_2_Hex_217-3257:14
- [Mate]: 0.5in Hex Shaft:16 ↔ 1_16_Acetal_Spacer_-_1_2_Hex_217-3257:14
- [Mate]: am-0150 Toughbox Large Output Gear:13 ↔ 1_16_Acetal_Spacer_-_1_2_Hex_217-3257:14
- [Mate]: 0.5in Hex Shaft:16 ↔ 18t_Aluminum_Spur_Gear_20_DP_1_2_Hex_Bore_217-3209:13
- [Mate]: 0.5in Hex Shaft:17 ↔ am-0150 Toughbox Large Output Gear:14
- [Mate]: 0.5in Hex Shaft:17 ↔ am-0150 Toughbox Large Output Gear:14
- [Mate]: 0.5in Hex Shaft:17 ↔ am-0150 Toughbox Large Output Gear:14
- [Mate]: 0.5in Hex Shaft:17 ↔ 18t_Aluminum_Spur_Gear_20_DP_1_2_Hex_Bore_217-3209:14
- [Mate]: 18t_Aluminum_Spur_Gear_20_DP_1_2_Hex_Bore_217-3209:14 ↔ am-0150 Toughbox Large Output Gear:14
- [Mate]: 0.5in Hex Shaft:17 ↔ 1_16_Acetal_Spacer_-_1_2_Hex_217-3257:15
- [Mate]: 0.5in Hex Shaft:17 ↔ 1_16_Acetal_Spacer_-_1_2_Hex_217-3257:15
- [Mate]: am-0150 Toughbox Large Output Gear:14 ↔ 1_16_Acetal_Spacer_-_1_2_Hex_217-3257:15
- [Mate]: 0.5in Hex Shaft:17 ↔ 18t_Aluminum_Spur_Gear_20_DP_1_2_Hex_Bore_217-3209:14
- Mate:240: am-0150 Toughbox Large Output Gear:11 ↔ 1_2_Acetal_Spacer_-_1_2_Hex_217-3261:16
- Mate:241: 0_500_ID_x_1_125_OD_x_0_313_WD_Flanged_Bearing_217-2731:11 ↔ 1_2_Acetal_Spacer_-_1_2_Hex_217-3261:16
- Mate:242: 1_2_Acetal_Spacer_-_1_2_Hex_217-3261:12 ↔ 0.5in Hex Shaft:15
- Mate:243: 1_2_Acetal_Spacer_-_1_2_Hex_217-3261:12 ↔ 0.5in Hex Shaft:15
- Mate:244: 1_2_Acetal_Spacer_-_1_2_Hex_217-3261:12 ↔ am-0150 Toughbox Large Output Gear:12
- Mate:245: 1_2_Acetal_Spacer_-_1_2_Hex_217-3261:14 ↔ 0.5in Hex Shaft:15
- Mate:246: 1_2_Acetal_Spacer_-_1_2_Hex_217-3261:14 ↔ 0.5in Hex Shaft:15
- Mate:247: 1_2_Acetal_Spacer_-_1_2_Hex_217-3261:12 ↔ 1_2_Acetal_Spacer_-_1_2_Hex_217-3261:14
- [Mate]: 0.5in Hex Shaft:18 ↔ am-0150 Toughbox Large Output Gear:15
- [Mate]: 0.5in Hex Shaft:18 ↔ am-0150 Toughbox Large Output Gear:15
- [Mate]: 0.5in Hex Shaft:18 ↔ am-0150 Toughbox Large Output Gear:15
- [Mate]: 0.5in Hex Shaft:18 ↔ 18t_Aluminum_Spur_Gear_20_DP_1_2_Hex_Bore_217-3209:15
- [Mate]: 18t_Aluminum_Spur_Gear_20_DP_1_2_Hex_Bore_217-3209:15 ↔ am-0150 Toughbox Large Output Gear:15
- [Mate]: 0.5in Hex Shaft:18 ↔ 18t_Aluminum_Spur_Gear_20_DP_1_2_Hex_Bore_217-3209:15
- [Mate]: 1_2_Acetal_Spacer_-_1_2_Hex_217-3261:17 ↔ 0.5in Hex Shaft:18
- [Mate]: 1_2_Acetal_Spacer_-_1_2_Hex_217-3261:17 ↔ 0.5in Hex Shaft:18
- [Mate]: 1_2_Acetal_Spacer_-_1_2_Hex_217-3261:17 ↔ am-0150 Toughbox Large Output Gear:15
- [Mate]: 1_2_Acetal_Spacer_-_1_2_Hex_217-3261:18 ↔ 0.5in Hex Shaft:18
- [Mate]: 1_2_Acetal_Spacer_-_1_2_Hex_217-3261:18 ↔ 0.5in Hex Shaft:18
- [Mate]: 1_2_Acetal_Spacer_-_1_2_Hex_217-3261:17 ↔ 1_2_Acetal_Spacer_-_1_2_Hex_217-3261:18
- [Mate]: 0.5in Hex Shaft:19 ↔ am-0150 Toughbox Large Output Gear:16
- [Mate]: 0.5in Hex Shaft:19 ↔ am-0150 Toughbox Large Output Gear:16
- [Mate]: 0.5in Hex Shaft:19 ↔ am-0150 Toughbox Large Output Gear:16
- [Mate]: 0.5in Hex Shaft:19 ↔ 18t_Aluminum_Spur_Gear_20_DP_1_2_Hex_Bore_217-3209:16
- [Mate]: 18t_Aluminum_Spur_Gear_20_DP_1_2_Hex_Bore_217-3209:16 ↔ am-0150 Toughbox Large Output Gear:16
- [Mate]: 0.5in Hex Shaft:19 ↔ 18t_Aluminum_Spur_Gear_20_DP_1_2_Hex_Bore_217-3209:16
- [Mate]: 1_2_Acetal_Spacer_-_1_2_Hex_217-3261:19 ↔ 0.5in Hex Shaft:19
- [Mate]: 1_2_Acetal_Spacer_-_1_2_Hex_217-3261:19 ↔ 0.5in Hex Shaft:19
- [Mate]: 1_2_Acetal_Spacer_-_1_2_Hex_217-3261:19 ↔ am-0150 Toughbox Large Output Gear:16
- [Mate]: 1_2_Acetal_Spacer_-_1_2_Hex_217-3261:20 ↔ 0.5in Hex Shaft:19
- [Mate]: 1_2_Acetal_Spacer_-_1_2_Hex_217-3261:20 ↔ 0.5in Hex Shaft:19
- [Mate]: 1_2_Acetal_Spacer_-_1_2_Hex_217-3261:19 ↔ 1_2_Acetal_Spacer_-_1_2_Hex_217-3261:20
- Mate:272: 0_500_ID_x_1_125_OD_x_0_313_WD_Flanged_Bearing_217-2731:10 ↔ 1_2_Acetal_Spacer_-_1_2_Hex_217-3261:14
## Named parameters: d203_d194 = 0 mm, d204_d195 = 0 mm, d205_d196 = 0 mm, d206_d198 = 0 mm, d207_d199 = 0 mm, d212_d203_d194 = 0 mm, d213_d204_d195 = 0 mm, d214_d205_d196 = 0 mm, d215_d206_d198 = 0 mm, d216_d207_d199 = 0 mm, d217_d209 = 0 mm, d218_d210 = 0 mm, d219_d211 = 0 mm, d223_d203_d194 = 0 mm, d224_d204_d195 = 0 mm, d225_d205_d196 = 0 mm, d226_d206_d198 = 0 mm, d227_d207_d199 = 0 mm, d235_d223_d203_d194 = 0 mm, d236_d224_d204_d195 = 0 mm, d237_d225_d205_d196 = 0 mm, d238_d226_d206_d198 = 0 mm, d239_d227_d207_d199 = 0 mm, d243_d232 = 0 mm, d244_d223_d203_d194 = 0 mm, d245_d224_d204_d195 = 0 mm, d246_d225_d205_d196 = 0 mm, d247_d226_d206_d198 = 0 mm, d248_d227_d207_d199 = 0 mm, d249_d228_d209 = 0 mm, d250_d229_d210 = 0 mm, d251_d230_d211 = 0 mm, d252_d232 = 0 mm, d253_d223_d203_d194 = 0 mm, d254_d224_d204_d195 = 0 mm, d255_d225_d205_d196 = 0 mm, d256_d226_d206_d198 = 0 mm, d257_d227_d207_d199 = 0 mm, d258_d228_d209 = 0 mm, d259_d229_d210 = 0 mm, d260_d230_d211 = 0 mm, d261_d232 = 0 mm, d270_d235_d223_d203_d194 = 0 mm, d271_d236_d224_d204_d195 = 0 mm, d272_d237_d225_d205_d196 = 0 mm, d273_d238_d226_d206_d198 = 0 mm, d274_d239_d227_d207_d199 = 0 mm, d275_d243_d232 = 0 mm, d276_d264 = 0 mm, d277_d265 = 0 mm, d278_d266 = 0 mm, d279_d267 = 0 mm, d280_d268 = 0 mm, d281_d269 = 0 mm, d282_d235_d223_d203_d194 = 0 mm, d283_d236_d224_d204_d195 = 0 mm, d284_d237_d225_d205_d196 = 0 mm, d285_d238_d226_d206_d198 = 0 mm, d286_d239_d227_d207_d199 = 0 mm, d287_d243_d232 = 0 mm, d288_d264 = 0 mm, d289_d265 = 0 mm, d290_d266 = 0 mm, d291_d267 = 0 mm, d292_d268 = 0 mm, d293_d269 = 0 mm
